# Autodesk Inventor assembly: GE-12096
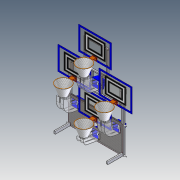
[picture p0: Inventor's stored thumbnail of the model, 180x180]
Saved by Autodesk Inventor 2012 (Build 160160000, 160)
## iProperties
Created: 2010-11-28
Part Number: GE-12096
Document SubType Name: Assembly
Designer: dfoster
Description: Basketball Hoop Assembly
Title: Basketball Hoop Assembly
Author: dfoster
## Documents named in this file (23)
- C:\Data Folder\FRC 2012 Field\Components\GE-12096.iam
- C:\Data Folder\FRC 2012 Field\Components\GE-12026.iam
- C:\Data Folder\FRC 2012 Field\Components\GE-12027.iam
- C:\Data Folder\FRC 2012 Field\Components\GE-12028.iam
- C:\Data Folder\FRC 2012 Field\Components\GE-12016.iam
- C:\Data Folder\FRC 2012 Field\Components\GE-12098.iam
- C:\Data Folder\FRC 2012 Field\Components\GE-12099.iam
- C:\Data Folder\FRC 2012 Field\Components\GE-12100.iam
- C:\Data Folder\FRC 2012 Field\Components\GE-12101.iam
- C:\Data Folder\FRC 2012 Field\Components\GE-12014.ipt
- C:\Data Folder\FRC 2012 Field\Components\GE-12072.iam
- C:\Data Folder\FRC 2012 Field\Components\GE-12088.iam
- C:\Data Folder\FRC 2012 Field\Components\GE-12059.ipt
- C:\Data Folder\FRC 2012 Field\Components\GE-12102.iam
- C:\Data Folder\FRC 2012 Field\Components\HW-00005.0005.ipt
- C:\Data Folder\FRC 2012 Field\Components\PP-00043.ipt
- C:\Data Folder\FRC 2012 Field\Components\HW-00063.ipt
- C:\Data Folder\FRC 2012 Field\Components\HW-00021.0001.ipt
- C:\Data Folder\FRC 2012 Field\Components\HW-00002.ipt
- C:\Data Folder\FRC 2012 Field\Components\HW-00073.ipt
- C:\Data Folder\FRC 2012 Field\Components\HW-00008.ipt
- C:\Data Folder\FRC 2012 Field\Components\HW-00011.0007.ipt
- C:\Data Folder\FRC 2012 Field\Components\HW-00015.ipt
## Components (140 placed, 22 different names)
1. GE-12026:1 [sub-assembly] — Flush:37, Flush:38, Mate:25, Flush:47, Tangent:18, Mate:29
2. GE-12027:1 [sub-assembly] — Flush:37, Flush:38, Mate:26
3. GE-12028:1 [sub-assembly] — Mate:25, Mate:26, Flush:44, Flush:45, Flush:46, Mate:51, Mate:52, Mate:53, Mate:54, Mate:55, Mate:56, Mate:57, Mate:58, Mate:59, Mate:63, Mate:64, Mate:65, Mate:66, Mate:67, Mate:68, Mate:69, Mate:70, Insert:23, Insert:25, Insert:26, Insert:27, Insert:28, Insert:29, Insert:30, Insert:39, Insert:40, Insert:47, Insert:50, Insert:51, Insert:52
4. GE-12016:2 [sub-assembly] — Flush:47, Tangent:18, Mate:29, Mate:32, Mate:33, Mate:34, Mate:35, Mate:36, Mate:37, Mate:38, Mate:39, Mate:40, Mate:41, Mate:42, Mate:43, Mate:48, Mate:49, Mate:50, Mate:60, Mate:61, Mate:62, Insert:4, Insert:5, Insert:6, Insert:7, Insert:8, Insert:17, Insert:18, Insert:19, Insert:20, Mate:74, Mate:75, Mate:76, Insert:21, Insert:22, Insert:24, Insert:48, Insert:49, Insert:53, Insert:54
5. GE-12098:1 [sub-assembly] — Mate:32, Mate:33, Mate:34, Flush:50, Mate:44, Insert:1, Flush:54
6. GE-12099:1 [sub-assembly] — Mate:35, Mate:36, Mate:37, Flush:51, Mate:45, Insert:2, Flush:55
7. GE-12100:1 [sub-assembly] — Mate:38, Mate:39, Mate:40, Flush:49, Mate:46, Insert:3, Flush:56
8. GE-12101:1 [sub-assembly] — Mate:41, Mate:42, Mate:43, Flush:52, Mate:47, Flush:57, Mate:77
9. GE-12014:1 — Flush:50, Mate:44
10. GE-12014:2 — Flush:51, Mate:45
11. GE-12014:3 — Flush:52, Mate:47
12. GE-12014:4 — Flush:49, Mate:46
13. GE-12072:1 [sub-assembly] — Mate:48, Mate:49, Mate:50, Insert:42, Insert:46
14. GE-12072:2 [sub-assembly] — Mate:54, Mate:55, Mate:56, Flush:53, Insert:37, Insert:43
15. GE-12072:3 [sub-assembly] — Mate:51, Mate:52, Mate:53, Insert:41, Insert:45
16. GE-12088:1 [sub-assembly] — Mate:57, Mate:58, Mate:59, Insert:38, Insert:44
17. GE-12059:1 — Mate:60, Mate:61, Mate:62, Flush:58, Flush:59, Mate:78, Mate:79
18. GE-12102:1 [sub-assembly] — Mate:63, Flush:53, Mate:66, Insert:33, Insert:34
19. GE-12102:2 [sub-assembly] — Mate:64, Mate:67, Mate:68, Insert:35, Insert:36
20. GE-12102:3 [sub-assembly] — Mate:65, Mate:69, Mate:70, Insert:31, Insert:32
21. HW-00063:1 — Insert:13
22. HW-00021.0001:1 — Insert:9, Insert:13
23. PP-00043:1 — Insert:5, Insert:9
24. HW-00002:1 — Insert:17
25. HW-00005.0005:1 — Insert:1
26. HW-00063:5
27. HW-00021.0001:5
28. PP-00043:5
29. HW-00002:5
30. HW-00005.0005:5
31. PP-00043:4 — Insert:6, Insert:10
32. HW-00021.0001:2 — Insert:10, Insert:14
33. HW-00063:2 — Insert:14
34. HW-00005.0005:2 — Insert:2
35. HW-00002:2 — Insert:18
36. PP-00043:3 — Insert:7, Insert:11
37. HW-00021.0001:3 — Insert:11, Insert:15
38. HW-00063:3 — Insert:15
39. HW-00005.0005:3 — Insert:3
40. HW-00002:3 — Insert:19
41. PP-00043:6
42. HW-00021.0001:6
43. HW-00063:6
44. HW-00005.0005:6
45. HW-00002:6
46. PP-00043:7
47. HW-00021.0001:7
48. HW-00063:7
49. HW-00005.0005:7
50. HW-00002:7
51. PP-00043:2 — Insert:8, Insert:12
52. HW-00021.0001:4 — Insert:12, Insert:16
53. HW-00063:4 — Insert:16
54. HW-00005.0005:4 — Insert:4
55. HW-00002:4 — Insert:20
56. PP-00043:8
57. HW-00021.0001:8
58. HW-00063:8
59. HW-00005.0005:8
60. HW-00002:8
61. HW-00008:1 — Flush:57, Mate:77
62. HW-00011.0007:3 — Insert:23
63. HW-00073:3 — Flush:54, Mate:74
64. HW-00011.0007:1 — Insert:21
65. HW-00008:2
66. HW-00011.0007:5
67. HW-00073:4
68. HW-00011.0007:6
69. HW-00073:1 — Flush:55, Mate:75
70. HW-00011.0007:2 — Insert:22
71. HW-00073:2 — Flush:56, Mate:76
72. HW-00011.0007:4 — Insert:24
73. HW-00073:5
74. HW-00011.0007:7
75. HW-00073:6
76. HW-00011.0007:8
77. HW-00015:1 — Insert:25
78. HW-00015:2 — Insert:27
79. HW-00015:3 — Insert:26
80. HW-00015:4 — Insert:28
81. HW-00015:5 — Insert:29
82. HW-00015:6 — Insert:30
83. HW-00002:9 — Insert:31
84. HW-00002:10 — Insert:32
85. HW-00002:11 — Insert:33
86. HW-00002:12 — Insert:35
87. HW-00002:13 — Insert:34
88. HW-00002:14 — Insert:36
89. HW-00015:7
90. HW-00015:8
91. HW-00015:9
92. HW-00015:10
93. HW-00015:11
94. HW-00015:12
95. HW-00002:15
96. HW-00002:16
97. HW-00002:17
98. HW-00002:18
99. HW-00002:19
100. HW-00002:20
101. HW-00015:13 — Insert:42
102. HW-00015:15 — Insert:44
103. HW-00015:17 — Insert:38
104. HW-00015:19 — Insert:37
105. HW-00015:21 — Insert:43
106. HW-00015:23 — Insert:41
107. HW-00015:25 — Insert:46
108. HW-00015:27 — Insert:45
109. HW-00002:21 — Insert:39
110. HW-00002:22 — Insert:47
111. HW-00002:23 — Insert:51
112. HW-00002:24 — Insert:50
113. HW-00002:25 — Insert:48
114. HW-00002:26 — Insert:52
115. HW-00002:27 — Insert:40
116. HW-00002:28 — Insert:49
117. HW-00015:28
118. HW-00015:29
119. HW-00015:30
120. HW-00015:31
121. HW-00015:32
122. HW-00015:33
123. HW-00015:34
124. HW-00015:35
125. HW-00002:29
126. HW-00002:30
127. HW-00002:31
128. HW-00002:32
129. HW-00002:33
130. HW-00002:34
131. HW-00002:35
132. HW-00002:36
133. HW-00073:7 — Flush:59, Mate:78
134. HW-00073:8 — Flush:58, Mate:79
135. HW-00011.0007:9 — Insert:54
136. HW-00011.0007:10 — Insert:53
137. HW-00073:9
138. HW-00073:10
139. HW-00011.0007:11
140. HW-00011.0007:12
## Component patterns: (2 elements, first: HW-00063:1 + HW-00021.0001:1 + PP-00043:1 + HW-00002:1 + HW-00005.0005:1), (2 elements, first: PP-00043:4 + HW-00021.0001:2 + HW-00063:2 + HW-00005.0005:2 + HW-00002:2 + PP-00043:3 + HW-00021.0001:3 + HW-00063:3 + HW-00005.0005:3 + HW-00002:3), (2 elements, first: PP-00043:2 + HW-00021.0001:4 + HW-00063:4 + HW-00005.0005:4 + HW-00002:4), (2 elements, first: HW-00008:1 + HW-00011.0007:3 + HW-00073:3 + HW-00011.0007:1), (2 elements, first: HW-00073:1 + HW-00011.0007:2 + HW-00073:2 + HW-00011.0007:4), (2 elements, first: HW-00015:1 + HW-00015:2 + HW-00015:3 + HW-00015:4 + HW-00015:5 + HW-00015:6 + HW-00002:9 + HW-00002:10 + HW-00002:11 + HW-00002:12 + HW-00002:13 + HW-00002:14), (2 elements, first: HW-00015:13 + HW-00015:15 + HW-00015:17 + HW-00015:19 + HW-00015:21 + HW-00015:23 + HW-00015:25 + HW-00015:27 + HW-00002:21 + HW-00002:22 + HW-00002:23 + HW-00002:24 + HW-00002:25 + HW-00002:26 + HW-00002:27 + HW-00002:28), (2 elements, first: HW-00073:7 + HW-00073:8 + HW-00011.0007:9 + HW-00011.0007:10)
## Relationships (120: Insert 54, Mate 48, Flush 17, Tangent 1)
- Flush:37: GE-12026:1 ↔ GE-12027:1
- Flush:38: GE-12026:1 ↔ GE-12027:1
- Mate:25 (3.175 mm): GE-12026:1 ↔ GE-12028:1
- Mate:26 (3.175 mm): GE-12027:1 ↔ GE-12028:1
- Flush:44: GE-12028:1
- Flush:45: GE-12028:1
- Flush:46: GE-12028:1
- Flush:47: GE-12026:1 ↔ GE-12016:2
- Tangent:18: GE-12026:1 ↔ GE-12016:2
- Mate:29 (3.175 mm): GE-12026:1 ↔ GE-12016:2
- Mate:32: GE-12016:2 ↔ GE-12098:1
- Mate:33: GE-12016:2 ↔ GE-12098:1
- Mate:34: GE-12016:2 ↔ GE-12098:1
- Mate:35: GE-12016:2 ↔ GE-12099:1
- Mate:36: GE-12016:2 ↔ GE-12099:1
- Mate:37: GE-12016:2 ↔ GE-12099:1
- Mate:38: GE-12016:2 ↔ GE-12100:1
- Mate:39: GE-12016:2 ↔ GE-12100:1
- Mate:40: GE-12016:2 ↔ GE-12100:1
- Mate:41: GE-12016:2 ↔ GE-12101:1
- Mate:42: GE-12016:2 ↔ GE-12101:1
- Mate:43: GE-12016:2 ↔ GE-12101:1
- Flush:49 (15.875 mm): GE-12100:1 ↔ GE-12014:4
- Flush:50 (15.875 mm): GE-12098:1 ↔ GE-12014:1
- Flush:51 (15.875 mm): GE-12099:1 ↔ GE-12014:2
- Flush:52 (15.875 mm): GE-12101:1 ↔ GE-12014:3
- Mate:44: GE-12098:1 ↔ GE-12014:1
- Mate:45: GE-12099:1 ↔ GE-12014:2
- Mate:46: GE-12100:1 ↔ GE-12014:4
- Mate:47: GE-12101:1 ↔ GE-12014:3
- Mate:48 (1.5875 mm): GE-12016:2 ↔ GE-12072:1
- Mate:49: GE-12016:2 ↔ GE-12072:1
- Mate:50: GE-12016:2 ↔ GE-12072:1
- Mate:51 (1.5875 mm): GE-12028:1 ↔ GE-12072:3
- Mate:52: GE-12028:1 ↔ GE-12072:3
- Mate:53: GE-12028:1 ↔ GE-12072:3
- Mate:54 (1.5875 mm): GE-12028:1 ↔ GE-12072:2
- Mate:55: GE-12028:1 ↔ GE-12072:2
- Mate:56: GE-12028:1 ↔ GE-12072:2
- Mate:57 (1.5875 mm): GE-12028:1 ↔ GE-12088:1
- Mate:58: GE-12028:1 ↔ GE-12088:1
- Mate:59: GE-12028:1 ↔ GE-12088:1
- Mate:60 (3.175 mm): GE-12016:2 ↔ GE-12059:1
- Mate:61: GE-12016:2 ↔ GE-12059:1
- Mate:62: GE-12016:2 ↔ GE-12059:1
- Mate:63: GE-12028:1 ↔ GE-12102:1
- Mate:64: GE-12028:1 ↔ GE-12102:2
- Mate:65: GE-12028:1 ↔ GE-12102:3
- Flush:53 (-1.5875 mm): GE-12072:2 ↔ GE-12102:1
- Mate:66: GE-12028:1 ↔ GE-12102:1
- Mate:67: GE-12028:1 ↔ GE-12102:2
- Mate:68: GE-12028:1 ↔ GE-12102:2
- Mate:69: GE-12028:1 ↔ GE-12102:3
- Mate:70: GE-12028:1 ↔ GE-12102:3
- Insert:1: GE-12098:1 ↔ HW-00005.0005:1
- Insert:2: GE-12099:1 ↔ HW-00005.0005:2
- Insert:3: GE-12100:1 ↔ HW-00005.0005:3
- Insert:4: GE-12016:2 ↔ HW-00005.0005:4
- Insert:5: GE-12016:2 ↔ PP-00043:1
- Insert:6: GE-12016:2 ↔ PP-00043:4
- Insert:7: GE-12016:2 ↔ PP-00043:3
- Insert:8: GE-12016:2 ↔ PP-00043:2
- Insert:9: HW-00021.0001:1 ↔ PP-00043:1
- Insert:10: PP-00043:4 ↔ HW-00021.0001:2
- Insert:11: PP-00043:3 ↔ HW-00021.0001:3
- Insert:12: PP-00043:2 ↔ HW-00021.0001:4
- Insert:13: HW-00063:1 ↔ HW-00021.0001:1
- Insert:14: HW-00021.0001:2 ↔ HW-00063:2
- Insert:15: HW-00021.0001:3 ↔ HW-00063:3
- Insert:16: HW-00021.0001:4 ↔ HW-00063:4
- Insert:17: GE-12016:2 ↔ HW-00002:1
- Insert:18: GE-12016:2 ↔ HW-00002:2
- Insert:19: GE-12016:2 ↔ HW-00002:3
- Insert:20: GE-12016:2 ↔ HW-00002:4
- Flush:54: GE-12098:1 ↔ HW-00073:3
- Mate:74: GE-12016:2 ↔ HW-00073:3
- Flush:55: GE-12099:1 ↔ HW-00073:1
- Mate:75: GE-12016:2 ↔ HW-00073:1
- Flush:56: GE-12100:1 ↔ HW-00073:2
- Mate:76: GE-12016:2 ↔ HW-00073:2
- Flush:57: GE-12101:1 ↔ HW-00008:1
- Mate:77: GE-12101:1 ↔ HW-00008:1
- Insert:21: GE-12016:2 ↔ HW-00011.0007:1
- Insert:22: GE-12016:2 ↔ HW-00011.0007:2
- Insert:23: GE-12028:1 ↔ HW-00011.0007:3
- Insert:24: GE-12016:2 ↔ HW-00011.0007:4
- Insert:25: GE-12028:1 ↔ HW-00015:1
- Insert:26: GE-12028:1 ↔ HW-00015:3
- Insert:27: GE-12028:1 ↔ HW-00015:2
- Insert:28: GE-12028:1 ↔ HW-00015:4
- Insert:29: GE-12028:1 ↔ HW-00015:5
- Insert:30: GE-12028:1 ↔ HW-00015:6
- Insert:31: GE-12102:3 ↔ HW-00002:9
- Insert:32: GE-12102:3 ↔ HW-00002:10
- Insert:33: GE-12102:1 ↔ HW-00002:11
- Insert:34: GE-12102:1 ↔ HW-00002:13
- Insert:35: GE-12102:2 ↔ HW-00002:12
- Insert:36: GE-12102:2 ↔ HW-00002:14
- Insert:37: GE-12072:2 ↔ HW-00015:19
- Insert:38: GE-12088:1 ↔ HW-00015:17
- Insert:39: GE-12028:1 ↔ HW-00002:21
- Insert:40: GE-12028:1 ↔ HW-00002:27
- Insert:41: GE-12072:3 ↔ HW-00015:23
- Insert:42: GE-12072:1 ↔ HW-00015:13
- Insert:43: GE-12072:2 ↔ HW-00015:21
- Insert:44: GE-12088:1 ↔ HW-00015:15
- Insert:45: GE-12072:3 ↔ HW-00015:27
- Insert:46: GE-12072:1 ↔ HW-00015:25
- Insert:47: GE-12028:1 ↔ HW-00002:22
- Insert:48: GE-12016:2 ↔ HW-00002:25
- Insert:49: GE-12016:2 ↔ HW-00002:28
- Insert:50: GE-12028:1 ↔ HW-00002:24
- Insert:51: GE-12028:1 ↔ HW-00002:23
- Insert:52: GE-12028:1 ↔ HW-00002:26
- Flush:58: GE-12059:1 ↔ HW-00073:8
- Flush:59: GE-12059:1 ↔ HW-00073:7
- Mate:78: GE-12059:1 ↔ HW-00073:7
- Mate:79: GE-12059:1 ↔ HW-00073:8
- Insert:53: GE-12016:2 ↔ HW-00011.0007:10
- Insert:54: GE-12016:2 ↔ HW-00011.0007:9
